# Autodesk Inventor assembly: pnp-head-assembly
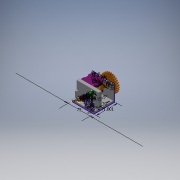
[picture p0: Inventor's stored thumbnail of the model, 180x180]
Saved by Autodesk Inventor 2017 (Build 210142000, 142)
## iProperties
Created: 2026-03-23
Part Number: pnp-head-assembly
Document SubType Name: Assembly
Designer: a
Author: a
## Documents named in this file (7)
- C:\Users\a\Documents\the-claw-pnp\cad\pnp-head-assembly.iam
- C:\Users\a\Documents\the-claw-pnp\cad\pnp-head.ipt
- C:\Users\a\Documents\the-claw-pnp\cad\vacuum-nozzle-assembly.iam
- C:\Users\a\Documents\the-claw-pnp\cad\gear-assembly.iam
- C:\Users\a\Documents\the-claw-pnp\cad\literally-just-a-cylinder-for-assembly-mockup-(silicone-sleeve).ipt
- C:\Users\a\Documents\the-claw-pnp\cad\3mm-nozzle-assembly.iam
- C:\Users\a\Documents\the-claw-pnp\cad\misc-models\17HS4401.ipt
## Components (6 placed, 6 different names)
1. pnp-head:1 — Mate:6, Mate:7, Mate:8, Mate:9, Mate:14, Flush:1, Flush:2
2. vacuum-nozzle-assembly:1 [sub-assembly] — Mate:6, Mate:7, Mate:10, Mate:11
3. gear-assembly:1 [sub-assembly] — Mate:8, Mate:9
4. literally-just-a-cylinder-for-assembly-mockup-(silicone-sleeve):1 — Mate:10, Mate:11, Mate:12, Mate:13
5. 3mm-nozzle-assembly:1 [sub-assembly] — Mate:12, Mate:13
6. 17HS4401:1 — Mate:14, Flush:1, Flush:2
## Relationships (11: Mate 9, Flush 2)
- Mate:6: pnp-head:1 ↔ vacuum-nozzle-assembly:1
- Mate:7: pnp-head:1 ↔ vacuum-nozzle-assembly:1
- Mate:8: pnp-head:1 ↔ gear-assembly:1
- Mate:9: pnp-head:1 ↔ gear-assembly:1
- Mate:10: vacuum-nozzle-assembly:1 ↔ literally-just-a-cylinder-for-assembly-mockup-(silicone-sleeve):1
- Mate:11: vacuum-nozzle-assembly:1 ↔ literally-just-a-cylinder-for-assembly-mockup-(silicone-sleeve):1
- Mate:12: literally-just-a-cylinder-for-assembly-mockup-(silicone-sleeve):1 ↔ 3mm-nozzle-assembly:1
- Mate:13: literally-just-a-cylinder-for-assembly-mockup-(silicone-sleeve):1 ↔ 3mm-nozzle-assembly:1
- Mate:14: pnp-head:1 ↔ 17HS4401:1
- Flush:1: pnp-head:1 ↔ 17HS4401:1
- Flush:2: pnp-head:1 ↔ 17HS4401:1
